# Autodesk Inventor assembly: linear-guide-Hand
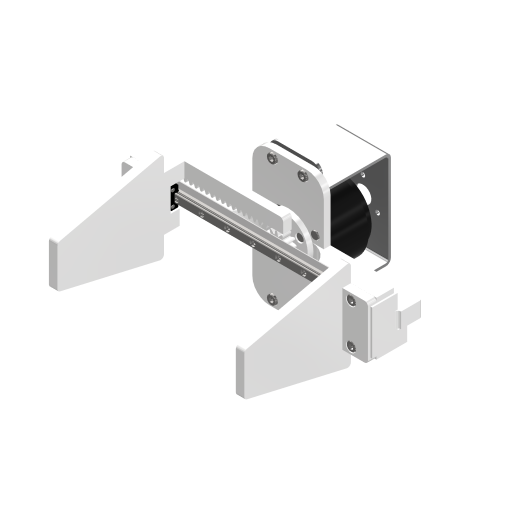
[picture p0: Inventor's stored thumbnail of the model, 512x512]
Saved by Autodesk Inventor 2023 (Build 270158000, 158)
## iProperties
Category: PARTsolutions
Company: MISUMI
Created: 2024-12-17
Part Number: linear-guide-Hand
Catalog Web Link: www.cadenas.de
Description: SSEB, SSEB-MX, SSE2B, SSE2B-MX, RSEB, RSE2B-Miniature Linear Guides Standard Blocks/Light Preload High Grade-L Selectable Type
Vendor: MISUMI
Document SubType Name: Assembly
Designer: psAdmin
Manufacturer: MISUMI
Mass: 135.965 g
Surface Area: 614.146 cm^2
Volume: 83.3375 cm^3
Density: 1.63149 g/cm^3
PSOL_IDENT_0: {$CADENAS_DATA/23d-libs/misumi/metric/06_linear_guides/re2b_asmtab.prj},256 {VTYP=3D},{STYP=ASSTAB},
PSOL_IDENT_1: {NB=SSE2B6-145},{LINA=SSE2B6-145},{NN=SSEB, SSEB-MX, SSE2B, SSE2B-MX, RSEB, RSE2B},{DATE=04.04.2024
PSOL_IDENT_2: 07:12:35},{GEOMDATE=07.03.2024 00:33:43},{VERSION=},{LINEID=60},{WBVAR=ST,MAT,MX,NOB,GREASE,LS,ALT1,
PSOL_IDENT_3: ALT2,ALT3,ALT4},{WBNUMERIC=LS}  {NB=SSE2B6-145},{LINA=SSE2B6-145},{KT=DUMMY},{PN=SSE2B6-145},{RT=B},
PSOL_IDENT_4: {TYPE=SSE2B},{ST=S},{MAT=S},{MX=},{MXALG= '','w/o MX(Lubrication unit)' },{NOB=2},{H=6},{GREASE=},{G
PSOL_IDENT_5: REASEALG='','Normal', 'L'  , 'L Type Greased ', 'G', 'G Type Greased', 'Y', 'Y Type Greased', 'H', '
PSOL_IDENT_6: H Type Greased'},{LT=Selectable},{LS=145},{HARD=56HRC~},{W=12},{L1=17.4},{B=8},{C=0},{SLL=M2x1.5},{L
PSOL_IDENT_7: 2=9.7},{K=4.5},{CBB=0.3},{W1=5},{W2=3.5},{H1=4.0},{CAA=0.3},{DD1DD2HH=2.4x3.5x1},{F=15},{G=5.0},{ALT
PSOL_IDENT_8: 1=},{ALT1ALG= '', 'w/o MC (Tapped Holes)' },{MC=M2.6},{ALT2=},{ALT2L=0.0},{ALT2N=0},{M=10},{LL=},{L0=
PSOL_IDENT_9: 70,85,100,115,130,145},{REC1=   '','Not applicable'    },{ST1='S', 'w/o Surface Treatment'},{MAT2='S'
PSOL_IDENT_10: ,'Stainless Steel'},{ALT3=},{ALT3ALG= '' , 'w/o WC (Pair of Rails)' , '-WC' , 'with WC (Set Pair of
PSOL_IDENT_11: Rails)' },{ALT4=},{ALT4ALG= '','N/A' },{PPATH=seb_series/seb_asmtpl.prj}
NB: SSE2B6-145
NN: SSEB, SSEB-MX, SSE2B, SSE2B-MX, RSEB, RSE2B
NT: Miniature Linear Guides Standard Blocks/Light Preload High Grade-L Selectable Type
NBSYN: $PN.
LINA: SSE2B6-145
CATALOG: Misumi
PN: SSE2B6-145
ST: w/o Surface Treatment
MAT: Stainless Steel
MX: w/o MX(Lubrication unit)
NOB: 2
H: 6
GREASE: Normal
LS: 145
W: 12
L1: 17.4
B: 8
C: 0
SLL: M2x1.5
L2: 9.7
K: 4.5
CBB: 0.3
W1: 5
W2: 3.5
H1: 4
CAA: 0.3
DD1DD2HH: 2.4x3.5x1
F: 15
G: 5
ALT1: w/o MC (Tapped Holes)
ALT2: Not applicable
ALT3: w/o WC (Pair of Rails)
ALT4: N/A
SUPPLIER: MISUMI
ARTICLENO: SSE2B6-145
BOMINFO: SSE2B6-145
CREATOR: CADENAS GmbH
Title: SSE2B6-145
Author: Cadenas PARTsolutions
Comments: Miniature Linear Guides Standard Blocks/Light Preload High Grade-L Selectable Type
## Documents named in this file (15)
- D:\GitHub\inventor\syu-si\OfficeRobot\Hand\linear-guide-Hand.iam
- D:\GitHub\inventor\syu-si\OfficeRobot\ReadyMade\linear_guide\SSE2B6-145\SSE2B6-145_r.ipt
- D:\GitHub\inventor\syu-si\OfficeRobot\ReadyMade\linear_guide\SSE2B6-145\SSEB6_b.ipt
- D:\GitHub\inventor\syu-si\OfficeRobot\ReadyMade\linear_guide\SSE2B6-145\M2x6_b.ipt
- D:\GitHub\inventor\syu-si\OfficeRobot\Hand\linear-gear.ipt
- D:\GitHub\inventor\syu-si\OfficeRobot\Hand\fix-guide-motor.ipt
- D:\GitHub\inventor\syu-si\OfficeRobot\Hand\hand-gear.ipt
- D:\GitHub\inventor\syu-si\OfficeRobot\ReadyMade\Steadywin\GIM3505-8_with-driver.ipt
- D:\GitHub\inventor\syu-si\OfficeRobot\ReadyMade\Screw\CSH-316L-M2_5-6.ipt
- D:\GitHub\inventor\syu-si\OfficeRobot\Hand\sheet.ipt
- D:\GitHub\inventor\syu-si\OfficeRobot\Hand\hand_box2.ipt
- D:\GitHub\inventor\syu-si\OfficeRobot\Hand\nail.ipt
- D:\GitHub\inventor\syu-si\OfficeRobot\ReadyMade\Screw\FB-305530.ipt
- D:\GitHub\inventor\syu-si\OfficeRobot\ReadyMade\Screw\CBE3-5.ipt
- D:\GitHub\inventor\syu-si\OfficeRobot\ReadyMade\Screw\FB-2001.ipt
## Components (42 placed, 14 different names)
1. linear-gear:1 — 挿入:66, 角度:4, メイト:18, 挿入:72, 挿入:73
2. fix-guide-motor:1 — メイト:14, 挿入:50, 挿入:51, 挿入:52, 挿入:53, 挿入:55, メイト:17, メイト:18
3. 平歯車1:1 — 角度:4
4. GIM3505-8_with-driver:1
5. CSH-316L-M2_5-6:1
6. CSH-316L-M2_5-6:2
7. CSH-316L-M2_5-6:3
8. sheet:1 — メイト:14, 挿入:54, 挿入:55, 挿入:56, 挿入:57
9. hand_box2:1 — フラッシュ:2
10. FB-305530:1 — 挿入:75
11. FB-305530:2 — 挿入:74
12. CBE3-5:1
13. CBE3-5:2
14. CBE3-5:3
15. CBE3-5:4
16. CBE3-5:7 — 挿入:76
17. CBE3-5:8 — 挿入:77
18. FB-2001:1 — 挿入:51
19. FB-2001:3 — 挿入:50
20. FB-2001:4 — 挿入:52
21. FB-2001:6 — 挿入:53, 挿入:54
22. CSH-316L-M2_5-6:4
23. CSH-316L-M2_5-6:5
24. CSH-316L-M2_5-6:6
25. SSE2B6-145_r:1 — 挿入:56, 挿入:57, 挿入:68, 挿入:69, 挿入:70, 挿入:71
26. SSEB6_b:1 — 挿入:66
27. SSEB6_b:2 — 挿入:67, 角度:3
28. M2x6_b:1 — 挿入:68
29. M2x6_b:2 — 挿入:69
30. M2x6_b:3 — 挿入:70
31. M2x6_b:4 — 挿入:71
32. linear-gear:2 — 挿入:67, メイト:17, 挿入:78, 挿入:79
33. nail:3 — 角度:3, フラッシュ:3
34. FB-305530:5
35. FB-305530:6
36. CBE3-5:9
37. CBE3-5:10
38. M2x6_b:5 — 挿入:73
39. M2x6_b:6 — 挿入:72
40. nail:4 — 挿入:74, 挿入:75, 挿入:76, 挿入:77
41. M2x6_b:7 — 挿入:78
42. M2x6_b:8 — 挿入:79
## Relationships (56: Insert 45, Mate 5, Angle 4, Flush 2)
- [Insert]: 平歯車1:1 ↔ GIM3505-8_with-driver:1
- [Insert]: fix-guide-motor:1 ↔ GIM3505-8_with-driver:1
- [Insert]: fix-guide-motor:1 ↔ GIM3505-8_with-driver:1
- [Insert]: fix-guide-motor:1 ↔ CSH-316L-M2_5-6:1
- [Insert]: fix-guide-motor:1 ↔ CSH-316L-M2_5-6:3
- [Insert]: fix-guide-motor:1 ↔ CSH-316L-M2_5-6:2
- [Insert]: fix-guide-motor:1 ↔ hand_box2:1
- [Insert]: fix-guide-motor:1 ↔ hand_box2:1
- [Insert]: linear-gear:1 ↔ FB-305530:2
- [Insert]: linear-gear:1 ↔ FB-305530:1
- [Insert]: fix-guide-motor:1 ↔ CBE3-5:2
- [Insert]: fix-guide-motor:1 ↔ CBE3-5:1
- [Insert]: fix-guide-motor:1 ↔ CBE3-5:3
- [Insert]: fix-guide-motor:1 ↔ CBE3-5:4
- [Insert]: 平歯車1:1 ↔ CSH-316L-M2_5-6:4
- [Insert]: 平歯車1:1 ↔ CSH-316L-M2_5-6:5
- [Insert]: 平歯車1:1 ↔ CSH-316L-M2_5-6:6
- メイト:14 [Mate]: fix-guide-motor:1 ↔ sheet:1
- 挿入:50 [Insert]: fix-guide-motor:1 ↔ FB-2001:3
- 挿入:51 [Insert]: fix-guide-motor:1 ↔ FB-2001:1
- 挿入:52 [Insert]: fix-guide-motor:1 ↔ FB-2001:4
- 挿入:53 [Insert]: fix-guide-motor:1 ↔ FB-2001:6
- 挿入:54 [Insert]: sheet:1 ↔ FB-2001:6
- [Mate]: SSE2B6-145_r:1 ↔ SSEB6_b:1
- [Angle] (0 deg): SSE2B6-145_r:1 ↔ SSEB6_b:1
- [Mate]: SSE2B6-145_r:1 ↔ SSEB6_b:2
- [Angle] (0 deg): SSE2B6-145_r:1 ↔ SSEB6_b:2
- 挿入:55 [Insert]: fix-guide-motor:1 ↔ sheet:1
- 挿入:56 [Insert]: sheet:1 ↔ SSE2B6-145_r:1
- 挿入:57 [Insert]: sheet:1 ↔ SSE2B6-145_r:1
- [Insert]: linear-gear:2 ↔ FB-305530:6
- [Insert]: linear-gear:2 ↔ FB-305530:5
- [Insert]: nail:3 ↔ FB-305530:5
- [Insert]: nail:3 ↔ FB-305530:6
- [Insert]: nail:3 ↔ CBE3-5:9
- [Insert]: nail:3 ↔ CBE3-5:10
- 挿入:66 [Insert]: linear-gear:1 ↔ SSEB6_b:1
- 挿入:67 [Insert]: SSEB6_b:2 ↔ linear-gear:2
- 角度:3 [Angle] (0 deg): SSEB6_b:2 ↔ nail:3
- 挿入:68 [Insert]: SSE2B6-145_r:1 ↔ M2x6_b:1
- 挿入:69 [Insert]: SSE2B6-145_r:1 ↔ M2x6_b:2
- 挿入:70 [Insert]: SSE2B6-145_r:1 ↔ M2x6_b:3
- 挿入:71 [Insert]: SSE2B6-145_r:1 ↔ M2x6_b:4
- 角度:4 [Angle] (0 deg): linear-gear:1 ↔ 平歯車1:1
- メイト:17 [Mate]: fix-guide-motor:1 ↔ linear-gear:2
- メイト:18 [Mate]: linear-gear:1 ↔ fix-guide-motor:1
- フラッシュ:2 [Flush] (28.5 mm): hand_box2:1
- フラッシュ:3 [Flush] (57.5 mm): nail:3
- 挿入:72 [Insert]: linear-gear:1 ↔ M2x6_b:6
- 挿入:73 [Insert]: linear-gear:1 ↔ M2x6_b:5
- 挿入:74 [Insert]: FB-305530:2 ↔ nail:4
- 挿入:75 [Insert]: FB-305530:1 ↔ nail:4
- 挿入:76 [Insert]: CBE3-5:7 ↔ nail:4
- 挿入:77 [Insert]: CBE3-5:8 ↔ nail:4
- 挿入:78 [Insert]: linear-gear:2 ↔ M2x6_b:7
- 挿入:79 [Insert]: linear-gear:2 ↔ M2x6_b:8
## Named parameters: d33_d74 = 0 mm, d34_d75 = 0 mm, d45_d86 = 0 mm, d46_d87 = 0 mm, d47_d88 = 0 mm, d60_d66 = 0 mm, d61_d67 = 0 mm, d66_d72 = 0 mm, d67_d73 = 0 mm, d140_d37_d78 = 0 mm, d141_d38_d79 = 0 mm, d142_d60_d66 = 0 mm, d143_d61_d67 = 0 mm, d144_d62_d68 = 0 mm, d145_d63_d69 = 0 mm
